# Autodesk Inventor assembly: AM14U3 Long
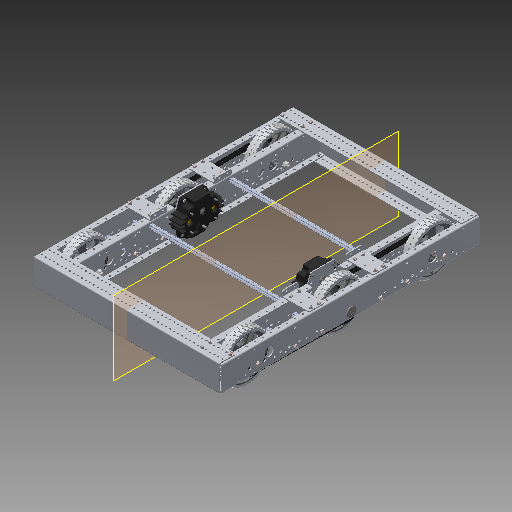
[picture p0: Inventor's stored thumbnail of the model, 512x512]
Saved by Autodesk Inventor 2018.2 (Build 222227000, 227)
## iProperties
Created: 2017-12-15
Part Number: AM14U3 Long
Document SubType Name: Assembly
Designer: PhillipD
Mass: 3792.36 g
Surface Area: 25550.9 cm^2
Volume: 3792.36 cm^3
Density: 1 g/cm^3
Author: PhillipD
Revision Number: ANY
## Documents named in this file (2)
- D:\snobotics\CAD-Development\robSteele\2018-FRC\AM14U3 Long with Bumper\Parts\AM14U3 Long.iam
- D:\snobotics\CAD-Development\robSteele\2018-FRC\AM14U3 Long with Bumper\Parts\AM14U3 Long Half.iam
## Components (2 placed, 2 different names)
1. AM14U3 Long Half_250 [sub-assembly]
2. AM14U3 Long Half_251 [sub-assembly] — Flush:1
## Relationships (1: Flush 1)
- Flush:1 (-298.45 mm): AM14U3 Long Half_251
